# Autodesk Inventor assembly: AssemblyTest
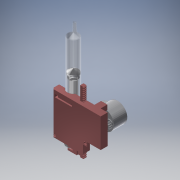
[picture p0: Inventor's stored thumbnail of the model, 180x180]
Saved by Autodesk Inventor 2018 (Build 220112000, 112)
## iProperties
Created: 2020-02-28
Part Number: AssemblyTest
Document SubType Name: Assembly
Designer: Ivan
Author: Ivan
## Documents named in this file (9)
- C:\Users\Ivan\Documents\GitHub\IdealGas\3D Model\Dependencies\AssemblyTest.iam
- C:\Users\Ivan\Documents\GitHub\IdealGas\3D Model\Dependencies\syringe_body.ipt
- C:\Users\Ivan\Documents\GitHub\IdealGas\3D Model\Dependencies\syringe_piston.ipt
- C:\Users\Ivan\Documents\GitHub\IdealGas\3D Model\Dependencies\syringe_plunger.ipt
- C:\Users\Ivan\Documents\GitHub\IdealGas\3D Model\Dependencies\Arm5.ipt
- C:\Users\Ivan\Documents\GitHub\IdealGas\3D Model\Dependencies\Base5.ipt
- C:\Users\Ivan\Documents\GitHub\IdealGas\3D Model\Dependencies\Rad3.ipt
- C:\Users\Ivan\Documents\GitHub\IdealGas\3D Model\Dependencies\Transm1.ipt
- C:\Users\Ivan\Documents\GitHub\IdealGas\3D Model\Dependencies\Geared Stepper.ipt
## Components (8 placed, 8 different names)
1. syringe_body:1 — Insert:2, Mate:1, Mate:2
2. syringe_plunger:1 — Insert:1, Insert:2, Angle:3
3. syringe_piston:1 — Insert:1
4. Arm5:1 — Angle:1, Mate:11, Mate:12
5. Base5:1 — Mate:1, Mate:2, Angle:1, Mate:7, Mate:8, Angle:2, Mate:9, Mate:10, Mate:11, Mate:12, Angle:3
6. Rad3:1 — Mate:5, Mate:6, Tangent:1
7. Transm1:1 — Mate:9, Mate:10
8. Geared Stepper:1 — Mate:5, Mate:6, Tangent:1, Mate:7, Mate:8, Angle:2
## Relationships (16: Mate 10, Angle 3, Insert 2, Tangent 1)
- Insert:1: syringe_plunger:1 ↔ syringe_piston:1
- Insert:2 (-18.2183 mm): syringe_body:1 ↔ syringe_plunger:1
- Mate:1: syringe_body:1 ↔ Base5:1
- Mate:2: syringe_body:1 ↔ Base5:1
- Angle:1 (180 deg): Arm5:1 ↔ Base5:1
- Mate:5: Rad3:1 ↔ Geared Stepper:1
- Mate:6: Rad3:1 ↔ Geared Stepper:1
- Tangent:1: Rad3:1 ↔ Geared Stepper:1
- Mate:7: Base5:1 ↔ Geared Stepper:1
- Mate:8: Base5:1 ↔ Geared Stepper:1
- Angle:2 (0 deg): Base5:1 ↔ Geared Stepper:1
- Mate:9: Base5:1 ↔ Transm1:1
- Mate:10: Base5:1 ↔ Transm1:1
- Mate:11: Arm5:1 ↔ Base5:1
- Mate:12: Arm5:1 ↔ Base5:1
- Angle:3 (0 deg): syringe_plunger:1 ↔ Base5:1
